# Autodesk Inventor assembly: am-0940
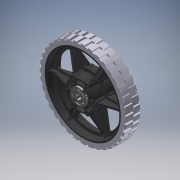
[picture p0: Inventor's stored thumbnail of the model, 180x180]
Saved by Autodesk Inventor 2017.1 (Build 211199000, 199)
## iProperties
Category: Loose Items
Company: Autodesk Inc.
Created: 2016-12-21
Part Number: am-0940
Document SubType Name: Assembly
Designer: Autodesk Inc.
Catalog Web Link: http://www.andymark.com/product-p/am-0940.htm
Vendor: AndyMark Inc.
Mass: 226.796 g
Surface Area: 1150.49 cm^2
Volume: 196.611 cm^3
Author: Autodesk Inc.
Keywords: Drive Base Kit
## Documents named in this file (4)
- D:\FIRST\FIRST KOP 2017\FIRST 2017 Drive Base Kit\am-0940.iam
- D:\FIRST\FIRST KOP 2017\FIRST 2017 Drive Base Kit\Parts\6 HiGrip Tread.ipt
- D:\FIRST\FIRST KOP 2017\FIRST 2017 Drive Base Kit\Parts\6in 2008 FIRST Hub.ipt
- D:\FIRST\FIRST KOP 2017\FIRST 2017 Drive Base Kit\Parts\DBK_1614ZZBearing_am-0209.ipt
## Components (4 placed, 3 different names)
1. 6 HiGrip Tread:1
2. 6in 2008 FIRST Hub:1 — Insert:1, Insert:2
3. DBK_1614ZZBearing_am-0209:1 — Insert:2
4. DBK_1614ZZBearing_am-0209:2 — Insert:1
## Relationships (2: Insert 2)
- Insert:1: 6in 2008 FIRST Hub:1 ↔ DBK_1614ZZBearing_am-0209:2
- Insert:2: 6in 2008 FIRST Hub:1 ↔ DBK_1614ZZBearing_am-0209:1
